# Autodesk Inventor assembly: Assembly1
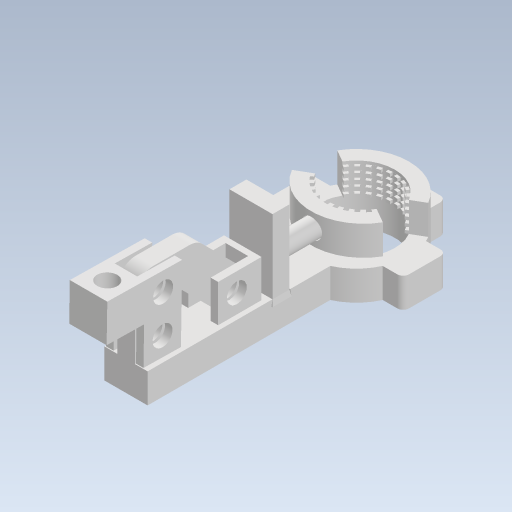
[picture p0: Inventor's stored thumbnail of the model, 512x512]
Saved by Autodesk Inventor 2023 (Build 270158000, 158)
## iProperties
Created: 2022-09-14
Part Number: Assembly1
Document SubType Name: Assembly
Designer: Dave
Author: Dave
## Documents named in this file (7)
- C:\Users\Dave\Desktop\Assembly1.iam
- C:\Users\Dave\Desktop\Plunger Cap.ipt
- C:\Users\Dave\Desktop\Plunger.ipt
- C:\Users\Dave\Desktop\Slider.ipt
- C:\Users\Dave\Desktop\Support Hole.ipt
- C:\Users\Dave\Desktop\Tensioner.ipt
- C:\Users\Dave\Desktop\Locker.ipt
## Components (6 placed, 6 different names)
1. Plunger Cap:1 — Mate:4, Angle:1, Tangent:1
2. Plunger:1 — Mate:3, Mate:4, Tangent:1, Angle:2, Mate:5, Mate:6
3. Slider:1 — Flush:1, Mate:1, Mate:2, Angle:1, Angle:2, Mate:9
4. Support Hole:1 — Flush:1, Mate:1, Mate:2, Mate:3
5. Tensioner:1 — Mate:5, Mate:6, Mate:7, Mate:8
6. Locker:1 — Mate:7, Mate:8, Mate:9
## Relationships (13: Mate 9, Angle 2, Flush 1, Tangent 1)
- Flush:1: Slider:1 ↔ Support Hole:1
- Mate:1: Slider:1 ↔ Support Hole:1
- Mate:2: Slider:1 ↔ Support Hole:1
- Mate:3: Plunger:1 ↔ Support Hole:1
- Mate:4: Plunger Cap:1 ↔ Plunger:1
- Angle:1 (0 deg): Plunger Cap:1 ↔ Slider:1
- Tangent:1: Plunger Cap:1 ↔ Plunger:1
- Angle:2 (0 deg): Plunger:1 ↔ Slider:1
- Mate:5: Plunger:1 ↔ Tensioner:1
- Mate:6 (0.81 mm): Plunger:1 ↔ Tensioner:1
- Mate:7: Tensioner:1 ↔ Locker:1
- Mate:8 (0.81 mm): Tensioner:1 ↔ Locker:1
- Mate:9: Slider:1 ↔ Locker:1
